# Autodesk Inventor assembly: chwytak
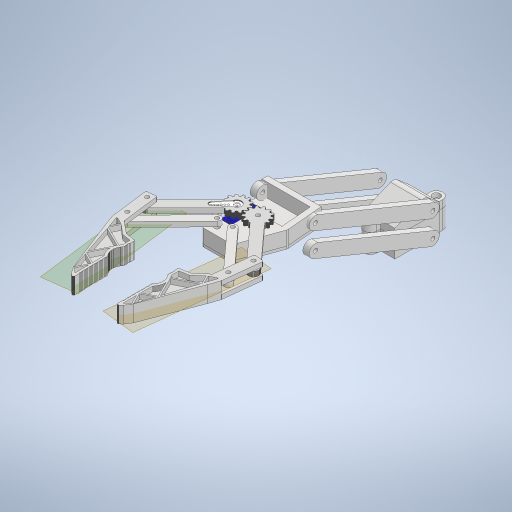
[picture p0: Inventor's stored thumbnail of the model, 512x512]
Saved by Autodesk Inventor 2023 (Build 270158000, 158)
## iProperties
Created: 2024-05-12
Part Number: chwytak
Document SubType Name: Assembly
Designer: kamil
Author: kamil
## Documents named in this file (12)
- C:\Users\kamil\Documents\PROJECTS - repos\ModBot---Projekt-Zespolowy\mechanics\modul_chwytaka\chwytak.iam
- C:\Users\kamil\Documents\PROJECTS - repos\ModBot---Projekt-Zespolowy\mechanics\modul_chwytaka\belka.ipt
- C:\Users\kamil\Documents\PROJECTS - repos\ModBot---Projekt-Zespolowy\mechanics\modul_chwytaka\Towerpro Micro Servo 9g.ipt
- C:\Users\kamil\Documents\PROJECTS - repos\ModBot---Projekt-Zespolowy\mechanics\modul_chwytaka\A1.ipt
- C:\Users\kamil\Documents\PROJECTS - repos\ModBot---Projekt-Zespolowy\mechanics\modul_chwytaka\uchwyt_serwa.ipt
- C:\Users\kamil\Documents\PROJECTS - repos\ModBot---Projekt-Zespolowy\mechanics\modul_chwytaka\belka_2.ipt
- C:\Users\kamil\Documents\PROJECTS - repos\ModBot---Projekt-Zespolowy\mechanics\modul_chwytaka\uchwyt_gorny.ipt
- C:\Users\kamil\Documents\PROJECTS - repos\ModBot---Projekt-Zespolowy\mechanics\modul_chwytaka\base_edited.ipt
- C:\Users\kamil\Documents\PROJECTS - repos\ModBot---Projekt-Zespolowy\mechanics\modul_chwytaka\Servo_Connector_Gear.ipt
- C:\Users\kamil\Documents\PROJECTS - repos\ModBot---Projekt-Zespolowy\mechanics\modul_chwytaka\Claw.ipt
- C:\Users\kamil\Documents\PROJECTS - repos\ModBot---Projekt-Zespolowy\mechanics\modul_chwytaka\Connector_Gear.ipt
- C:\Users\kamil\Documents\PROJECTS - repos\ModBot---Projekt-Zespolowy\mechanics\modul_chwytaka\conector.ipt
## Components (17 placed, 11 different names)
1. belka:1 — Zestawiające:4, Zestawiające:5, Kątowe:1, Zestawiające:12, Równoległe:3
2. Towerpro Micro Servo 9g:1 — Zestawiające:1, Zestawiające:2, Równoległe:1, Zestawiające:3, Zestawiające:6, Zestawiające:7, Zestawiające:8, Zestawiające:9, Kątowe:4
3. A1:1 — Zestawiające:2, Zestawiające:3, Zestawiające:4, Zestawiające:5, Kątowe:1
4. uchwyt_serwa:1 — Zestawiające:7, Zestawiające:8, Zestawiające:9, Zestawiające:10, Zestawiające:11, Zestawiające:13, Zestawiające:14, Zestawiające:15, Kątowe:5
5. belka_2:1 — Zestawiające:10, Zestawiające:11, Zestawiające:12, Równoległe:2, Kątowe:2
6. uchwyt_gorny:1 — Zestawiające:13, Zestawiające:14, Zestawiające:15, Zestawiające:16, Zestawiające:17
7. belka_2:2 — Zestawiające:16, Równoległe:2, Kątowe:2, Równoległe:4, Zestawiające:44
8. belka_2:3 — Zestawiające:17, Równoległe:3, Równoległe:4
9. base_edited:1 — Zestawiające:24, Zestawiające:25, Zestawiające:35, Zestawiające:36, Zestawiające:37, Zestawiające:38, Kątowe:4, Kątowe:5, Zestawiające:44
10. Servo_Connector_Gear:1 — Zestawiające:33, Zestawiające:34, Kątowe:3, Równoległe:5, Równoległe:7, Zestawiające:39, Zestawiające:43
11. Claw:1 — Zestawiające:39, Zestawiające:40, Równoległe:8, Zestawiające:43
12. Connector_Gear:1 — Zestawiające:35, Równoległe:5, Równoległe:6, Zestawiające:41
13. Towerpro Micro Servo 9g:2 — Zestawiające:24, Zestawiające:25, Zestawiające:27, Zestawiające:28, Zestawiające:36
14. A1:2 — Zestawiające:27, Zestawiające:28, Zestawiające:33, Zestawiające:34, Kątowe:3
15. conector:1 — Zestawiające:37, Równoległe:6, Zestawiające:42
16. conector:2 — Zestawiające:38, Równoległe:7, Zestawiające:40
17. Claw:2 — Równoległe:8, Zestawiające:41, Zestawiające:42
## Relationships (46: Mate 33, Flush 8, Angle 5)
- Zestawiające:1 [Mate]: Towerpro Micro Servo 9g:1
- Zestawiające:2 [Mate]: Towerpro Micro Servo 9g:1 ↔ A1:1
- Równoległe:1 [Flush]: Towerpro Micro Servo 9g:1
- Zestawiające:3 [Mate]: Towerpro Micro Servo 9g:1 ↔ A1:1
- Zestawiające:4 [Mate]: belka:1 ↔ A1:1
- Zestawiające:5 [Mate]: belka:1 ↔ A1:1
- Kątowe:1 [Angle] (180 deg): belka:1 ↔ A1:1
- Zestawiające:6 [Mate]: Towerpro Micro Servo 9g:1
- Zestawiające:7 [Mate]: Towerpro Micro Servo 9g:1 ↔ uchwyt_serwa:1
- Zestawiające:8 [Mate] (0.5 mm): Towerpro Micro Servo 9g:1 ↔ uchwyt_serwa:1
- Zestawiające:9 [Mate]: Towerpro Micro Servo 9g:1 ↔ uchwyt_serwa:1
- Zestawiające:10 [Mate] (2 mm): uchwyt_serwa:1 ↔ belka_2:1
- Zestawiające:11 [Mate]: uchwyt_serwa:1 ↔ belka_2:1
- Zestawiające:12 [Mate]: belka:1 ↔ belka_2:1
- Zestawiające:13 [Mate]: uchwyt_serwa:1 ↔ uchwyt_gorny:1
- Zestawiające:14 [Mate]: uchwyt_serwa:1 ↔ uchwyt_gorny:1
- Zestawiające:15 [Mate]: uchwyt_serwa:1 ↔ uchwyt_gorny:1
- Zestawiające:16 [Mate]: uchwyt_gorny:1 ↔ belka_2:2
- Równoległe:2 [Flush]: belka_2:1 ↔ belka_2:2
- Kątowe:2 [Angle] (180 deg): belka_2:1 ↔ belka_2:2
- Zestawiające:17 [Mate]: uchwyt_gorny:1 ↔ belka_2:3
- Równoległe:3 [Flush]: belka:1 ↔ belka_2:3
- Równoległe:4 [Flush]: belka_2:2 ↔ belka_2:3
- Zestawiające:24 [Mate] (0.3 mm): base_edited:1 ↔ Towerpro Micro Servo 9g:2
- Zestawiające:25 [Mate]: base_edited:1 ↔ Towerpro Micro Servo 9g:2
- Zestawiające:27 [Mate]: Towerpro Micro Servo 9g:2 ↔ A1:2
- Zestawiające:28 [Mate]: Towerpro Micro Servo 9g:2 ↔ A1:2
- Zestawiające:33 [Mate]: Servo_Connector_Gear:1 ↔ A1:2
- Zestawiające:34 [Mate]: Servo_Connector_Gear:1 ↔ A1:2
- Kątowe:3 [Angle] (180 deg): Servo_Connector_Gear:1 ↔ A1:2
- Zestawiające:35 [Mate]: base_edited:1 ↔ Connector_Gear:1
- Równoległe:5 [Flush]: Servo_Connector_Gear:1 ↔ Connector_Gear:1
- Zestawiające:36 [Mate] (0.05 mm): base_edited:1 ↔ Towerpro Micro Servo 9g:2
- Zestawiające:37 [Mate]: base_edited:1 ↔ conector:1
- Zestawiające:38 [Mate]: base_edited:1 ↔ conector:2
- Równoległe:6 [Flush]: Connector_Gear:1 ↔ conector:1
- Równoległe:7 [Flush]: Servo_Connector_Gear:1 ↔ conector:2
- Zestawiające:39 [Mate]: Servo_Connector_Gear:1 ↔ Claw:1
- Zestawiające:40 [Mate]: Claw:1 ↔ conector:2
- Równoległe:8 [Flush]: Claw:1 ↔ Claw:2
- Zestawiające:41 [Mate]: Connector_Gear:1 ↔ Claw:2
- Zestawiające:42 [Mate]: conector:1 ↔ Claw:2
- Zestawiające:43 [Mate] (1 mm): Servo_Connector_Gear:1 ↔ Claw:1
- Kątowe:4 [Angle] (0 deg): Towerpro Micro Servo 9g:1 ↔ base_edited:1
- Kątowe:5 [Angle] (0 deg): uchwyt_serwa:1 ↔ base_edited:1
- Zestawiające:44 [Mate]: belka_2:2 ↔ base_edited:1
